# Autodesk Inventor assembly: INDX_000_Main
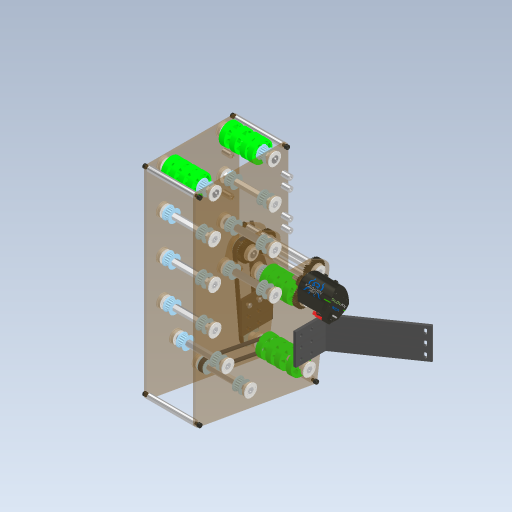
[picture p0: Inventor's stored thumbnail of the model, 512x512]
Saved by Autodesk Inventor 2024 (Build 280153000, 153)
## iProperties
Created: 2024-08-08
Part Number: INDX_000_Main
Document SubType Name: Assembly
Designer: Oscar
Author: Oscar
## Documents named in this file (27)
- C:\Users\Takum\OneDrive\Documents\GitHub\1622-2024-Summer-CAD-A-Thon\Index\INDX_000_Main.iam
- C:\Users\Takum\OneDrive\Documents\GitHub\1622-2024-Summer-CAD-A-Thon\Index\INDX_001_Plate.ipt
- C:\Users\Takum\OneDrive\Documents\GitHub\1622-2024-Summer-CAD-A-Thon\Index\INDX_002_Standoff.ipt
- C:\Users\Takum\OneDrive\Documents\GitHub\1622-2024-Summer-CAD-A-Thon\COTS Library\Motion\Bearings\COTS_WCP-0783_1.125ODHexBearing.ipt
- C:\Users\Takum\OneDrive\Documents\GitHub\1622-2024-Summer-CAD-A-Thon\COTS Library\Motors\COTS_WCP_Full_Kraken.iam
- C:\Users\Takum\OneDrive\Documents\GitHub\1622-2024-Summer-CAD-A-Thon\Index\INDX_003_OuterStandoff.ipt
- C:\Users\Takum\OneDrive\Documents\GitHub\1622-2024-Summer-CAD-A-Thon\Index\INDX_006_Funnel.ipt
- C:\Users\Takum\OneDrive\Documents\GitHub\1622-2024-Summer-CAD-A-Thon\COTS Library\Motion\Gears\Motor Gears\SplineXS\COTS_WCP-1013_14TSplineXsGear.ipt
- C:\Users\Takum\OneDrive\Documents\GitHub\1622-2024-Summer-CAD-A-Thon\COTS Library\Motion\Gears\20DP gears\Steel\0.5in hex\COTS_WCP-0174_Steel_34T20DPGear.ipt
- C:\Users\Takum\OneDrive\Documents\GitHub\1622-2024-Summer-CAD-A-Thon\Index\INDX_007_22TPulley.ipt
- C:\Users\Takum\OneDrive\Documents\GitHub\1622-2024-Summer-CAD-A-Thon\Index\INDX_008_0.5inSpacer.ipt
- C:\Users\Takum\OneDrive\Documents\GitHub\1622-2024-Summer-CAD-A-Thon\COTS Library\Motion\Wheels\Compliant Wheels\2in compliant wheels\0.500in hex bore\COTS_am-3462_2indiameter_0.500inhexbore_durometer35A_CompliantWheel.ipt
- C:\Users\Takum\OneDrive\Documents\GitHub\1622-2024-Summer-CAD-A-Thon\Index\INDX_010_5inHex.ipt
- C:\Users\Takum\OneDrive\Documents\GitHub\1622-2024-Summer-CAD-A-Thon\Index\INDX_011_SecondPlate.ipt
- C:\Users\Takum\OneDrive\Documents\GitHub\1622-2024-Summer-CAD-A-Thon\Index\INDX_012_OuterPlate.ipt
- C:\Users\Takum\OneDrive\Documents\GitHub\1622-2024-Summer-CAD-A-Thon\Index\INDX_013_ThinSpacer.ipt
- C:\Users\Takum\OneDrive\Documents\GitHub\1622-2024-Summer-CAD-A-Thon\Index\INDX_014_Outerstandoff.ipt
- C:\Users\Takum\OneDrive\Documents\GitHub\1622-2024-Summer-CAD-A-Thon\Index\INDX_009_FrontHex.ipt
- C:\Users\Takum\OneDrive\Documents\GitHub\1622-2024-Summer-CAD-A-Thon\Index\INDX_015_OuterHex.ipt
- C:\Users\Takum\OneDrive\Documents\GitHub\1622-2024-Summer-CAD-A-Thon\Index\INDX_016_BottomHex.ipt
- C:\Users\Takum\OneDrive\Documents\GitHub\1622-2024-Summer-CAD-A-Thon\COTS Library\Motion\Pulleys\HTD5M\10mm Wide\COTS_HTD5MM_9mm_16TPulley.ipt
- C:\Users\Takum\OneDrive\Documents\GitHub\1622-2024-Summer-CAD-A-Thon\Index\INDX_017_Mainhex.ipt
- C:\Users\Takum\OneDrive\Documents\GitHub\1622-2024-Summer-CAD-A-Thon\Index\INDX_021_BottomBelt.ipt
- C:\Users\Takum\OneDrive\Documents\GitHub\1622-2024-Summer-CAD-A-Thon\COTS Library\Fasteners\Washers\COTS_90107A029_316 Stainless Steel Washer.ipt
- C:\Users\Takum\OneDrive\Documents\GitHub\1622-2024-Summer-CAD-A-Thon\COTS Library\Fasteners\Bolts\Button-Head\0.25-20\COTS_0.25-20_ButtonHead_0.5inlong_StainlessSteel_92949A537.ipt
- C:\Users\Takum\OneDrive\Documents\GitHub\1622-2024-Summer-CAD-A-Thon\COTS Library\Fasteners\Bolts\Socket-Head\0.25-20\COTS_91251A540_Black-Oxide Alloy Steel Socket Head Screw.ipt
- C:\Users\Takum\OneDrive\Documents\GitHub\1622-2024-Summer-CAD-A-Thon\Index\INDX_022_SideBelt.ipt
## Components (159 placed, 26 different names)
1. INDX_001_Plate:2 — Mate:3, Mate:5, Mate:6, Mate:9, Mate:10, Mate:12, Mate:13, Mate:14, Mate:15, Mate:16, Mate:17, Mate:18, Mate:19, Mate:20, Mate:21, Mate:22, Mate:23, Mate:24, Mate:25, Mate:26, Mate:27, Mate:28, Mate:29, Mate:30, Mate:31, Mate:54, Mate:56, Mate:57, Mate:58, Mate:59, Mate:60, Mate:61, Mate:62, Mate:63, Mate:64, Mate:65, Mate:66, Mate:67, Mate:68, Mate:69, Mate:70, Mate:79, Mate:80, Mate:81, Mate:89, Mate:162, Mate:165, Mate:278, Mate:279, Mate:280, Mate:281, Mate:295, Mate:296, Mate:300, Mate:301
2. INDX_002_Standoff:1 — Mate:9, Mate:149, Mate:274
3. INDX_002_Standoff:2 — Mate:6, Mate:148, Mate:275
4. INDX_002_Standoff:3 — Mate:10, Mate:111, Mate:150
5. INDX_002_Standoff:4 — Mate:3, Mate:5, Mate:110, Mate:112
6. COTS_WCP-0783_1.125ODHexBearing:1 — Mate:18, Mate:19, Mate:264, Mate:265, Mate:311
7. COTS_WCP-0783_1.125ODHexBearing:2 — Mate:16, Mate:17, Mate:310
8. COTS_WCP-0783_1.125ODHexBearing:3 — Mate:20, Mate:21, Mate:318
9. COTS_WCP-0783_1.125ODHexBearing:4 — Mate:22, Mate:23, Mate:262, Mate:263, Mate:319
10. COTS_WCP-0783_1.125ODHexBearing:5 — Mate:13, Mate:14, Mate:307
11. COTS_WCP-0783_1.125ODHexBearing:6 — Mate:12, Mate:15, Mate:306
12. COTS_WCP-0783_1.125ODHexBearing:7 — Mate:24, Mate:25
13. COTS_WCP-0783_1.125ODHexBearing:8 — Mate:26, Mate:27
14. COTS_WCP-0783_1.125ODHexBearing:9 — Mate:30, Mate:31
15. COTS_WCP-0783_1.125ODHexBearing:10 — Mate:28, Mate:29
16. COTS_WCP-0783_1.125ODHexBearing:11 — Mate:140, Mate:141, Mate:194, Flush:11, Mate:216, Mate:217, Mate:308
17. COTS_WCP-0783_1.125ODHexBearing:12 — Mate:132, Mate:133, Mate:192, Flush:9, Mate:218, Mate:313, Mate:316
18. COTS_WCP-0783_1.125ODHexBearing:13 — Mate:134, Mate:135, Mate:242, Flush:16, Mate:288, Mate:317
19. COTS_WCP-0783_1.125ODHexBearing:14 — Mate:146, Mate:147, Mate:189, Flush:6, Mate:198, Mate:202, Mate:203, Mate:302
20. COTS_WCP-0783_1.125ODHexBearing:15 — Mate:130, Mate:131, Mate:191, Flush:8, Mate:212, Mate:314, Mate:315
21. COTS_WCP-0783_1.125ODHexBearing:16 — Mate:142, Mate:143, Mate:193, Flush:10, Mate:214, Mate:215, Mate:305
22. COTS_WCP-0783_1.125ODHexBearing:17 — Mate:144, Mate:145, Mate:190, Flush:7, Mate:204, Mate:205, Mate:303, Mate:304
23. COTS_WCP-0783_1.125ODHexBearing:18 — Mate:96, Mate:100, Mate:102, Mate:153, Mate:154
24. COTS_WCP-0783_1.125ODHexBearing:19 — Mate:138, Mate:139, Mate:196, Flush:13, Mate:286, Mate:309
25. COTS_WCP-0783_1.125ODHexBearing:20 — Mate:113, Mate:114, Mate:195, Flush:12, Mate:250, Mate:260, Mate:261
26. COTS_WCP-0783_1.125ODHexBearing:21 — Mate:136, Mate:137, Mate:197, Flush:14, Mate:254, Mate:258
27. COTS_WCP_Full_Kraken:1 [sub-assembly] — Mate:54, Mate:56, Mate:89, Mate:90
28. COTS_WCP-0783_1.125ODHexBearing:22 — Mate:59, Mate:60, Mate:91, Mate:92
29. COTS_WCP-0783_1.125ODHexBearing:23 — Mate:57, Mate:58, Mate:93, Mate:94
30. COTS_WCP-0783_1.125ODHexBearing:24 — Mate:61, Mate:62, Mate:184
31. INDX_003_OuterStandoff:1 — Mate:115, Mate:116
32. INDX_003_OuterStandoff:2 — Mate:119, Mate:120
33. INDX_003_OuterStandoff:3 — Mate:63, Mate:68
34. INDX_003_OuterStandoff:4 — Mate:64, Mate:69
35. INDX_003_OuterStandoff:5 — Mate:65, Mate:70
36. INDX_003_OuterStandoff:6 — Mate:66, Mate:67
37. INDX_003_OuterStandoff:7 — Mate:117, Mate:118
38. INDX_003_OuterStandoff:8 — Mate:121, Mate:122
39. INDX_006_Funnel:1 — Mate:79, Mate:80, Mate:81
40. INDX_006_Funnel:2 — Mate:123, Mate:124, Mate:125
41. COTS_WCP-0783_1.125ODHexBearing:25 — Mate:126, Mate:127, Mate:128, Mate:129
42. COTS_WCP-0783_1.125ODHexBearing:26 — Mate:109, Flush:2, Mate:151, Mate:152, Mate:210, Mate:312
43. COTS_WCP-1013_14TSplineXsGear:1 — Mate:90
44. COTS_WCP-0174_Steel_34T20DPGear:1 — Mate:93, Mate:94, Mate:108
45. COTS_WCP-0174_Steel_34T20DPGear:2 — Mate:91, Mate:92
46. INDX_007_22TPulley:1 — Mate:159, Mate:160, Mate:172, Mate:173, Mate:248, Mate:249
47. INDX_007_22TPulley:2 — Mate:96, Mate:101, Flush:5, Mate:220, Mate:247
48. INDX_008_0.5inSpacer:1 — Mate:100, Mate:101, Mate:102, Mate:183
49. COTS_am-3462_2indiameter_0.500inhexbore_durometer35A_CompliantWheel:1 — Mate:105
50. COTS_am-3462_2indiameter_0.500inhexbore_durometer35A_CompliantWheel:2 — Mate:106, Mate:107
51. COTS_am-3462_2indiameter_0.500inhexbore_durometer35A_CompliantWheel:3 — Mate:107
52. COTS_am-3462_2indiameter_0.500inhexbore_durometer35A_CompliantWheel:4 — Mate:105, Mate:106, Mate:108
53. INDX_010_5inHex:1 — Mate:109, Flush:2, Mate:211, Mate:234
54. INDX_011_SecondPlate:1 — Mate:110, Mate:111, Mate:112, Mate:113, Mate:114, Mate:115, Mate:116, Mate:117, Mate:118, Mate:119, Mate:120, Mate:121, Mate:122, Mate:123, Mate:124, Mate:125, Mate:126, Mate:127, Mate:130, Mate:131, Mate:132, Mate:133, Mate:134, Mate:135, Mate:136, Mate:137, Mate:138, Mate:139, Mate:140, Mate:141, Mate:142, Mate:143, Mate:144, Mate:145, Mate:146, Mate:147, Mate:148, Mate:149, Mate:150, Mate:151, Mate:152, Mate:153, Mate:154, Mate:155, Mate:156, Mate:157, Mate:163, Mate:164, Mate:166, Mate:167, Mate:175, Mate:177, Mate:179, Mate:243, Mate:244, Mate:245, Mate:246, Mate:276, Mate:277, Mate:294, Mate:297, Mate:298, Mate:299
55. COTS_WCP-0174_Steel_34T20DPGear:3 — Mate:128, Mate:129, Mate:181
56. COTS_WCP-0174_Steel_34T20DPGear:4 — Mate:155, Mate:158, Mate:159, Mate:160
57. COTS_WCP-0783_1.125ODHexBearing:27 — Mate:156, Mate:157, Mate:158, Mate:320
58. INDX_002_Standoff:5 — Mate:162, Mate:163
59. INDX_002_Standoff:6 — Mate:164, Mate:165
60. INDX_012_OuterPlate:1 — Mate:166, Mate:167, Mate:168, Mate:169, Mate:170, Mate:171, Mate:176, Mate:178, Mate:180, Mate:236, Mate:237, Mate:238, Mate:239
61. COTS_WCP-0783_1.125ODHexBearing:28 — Mate:170, Mate:171, Mate:174, Mate:182, Flush:4, Mate:208, Mate:209
62. COTS_WCP-0783_1.125ODHexBearing:29 — Mate:168, Mate:169, Flush:3, Mate:206, Mate:207
63. INDX_013_ThinSpacer:1 — Mate:172, Mate:173, Mate:174
64. INDX_014_Outerstandoff:1 — Mate:175, Mate:176
65. INDX_014_Outerstandoff:2 — Mate:177, Mate:178
66. INDX_014_Outerstandoff:3 — Mate:179, Mate:180
67. INDX_009_FrontHex:1 — Mate:181, Flush:3, Mate:232
68. INDX_015_OuterHex:1 — Mate:182, Flush:4, Mate:230, Mate:321, Mate:322
69. INDX_016_BottomHex:1 — Mate:183, Flush:5, Mate:221, Mate:222
70. COTS_am-3462_2indiameter_0.500inhexbore_durometer35A_CompliantWheel:5 — Mate:184, Mate:185, Mate:186
71. COTS_am-3462_2indiameter_0.500inhexbore_durometer35A_CompliantWheel:6 — Mate:185
72. COTS_am-3462_2indiameter_0.500inhexbore_durometer35A_CompliantWheel:7 — Mate:186, Mate:187, Mate:188
73. COTS_am-3462_2indiameter_0.500inhexbore_durometer35A_CompliantWheel:8 — Mate:187
74. COTS_HTD5MM_9mm_16TPulley:1 — Mate:188, Flush:15, Mate:199
75. INDX_017_Mainhex:1 — Mate:190, Flush:7, Mate:226
76. INDX_017_Mainhex:2 — Mate:189, Flush:6, Mate:224
77. INDX_017_Mainhex:3 — Mate:192, Flush:9, Mate:219, Mate:240
78. INDX_017_Mainhex:4 — Mate:193, Flush:10, Mate:284
79. INDX_017_Mainhex:5 — Mate:191, Flush:8, Mate:213, Mate:228
80. INDX_017_Mainhex:6 — Mate:194, Flush:11, Mate:282
81. INDX_017_Mainhex:7 — Mate:195, Flush:12, Mate:270
82. INDX_017_Mainhex:8 — Mate:196, Flush:13, Mate:287, Mate:292
83. INDX_017_Mainhex:9 — Mate:197, Flush:14, Mate:259, Mate:272
84. COTS_HTD5MM_9mm_16TPulley:2 — Mate:198, Flush:15, Mate:200, Mate:201
85. INDX_021_BottomBelt:1 — Mate:199, Mate:200, Mate:201
86. COTS_90107A029_316 Stainless Steel Washer:1 — Mate:202, Mate:203, Mate:225
87. COTS_90107A029_316 Stainless Steel Washer:2 — Mate:204, Mate:205, Mate:227
88. COTS_90107A029_316 Stainless Steel Washer:3 — Mate:206, Mate:207, Mate:233
89. COTS_90107A029_316 Stainless Steel Washer:4 — Mate:208, Mate:209, Mate:231
90. COTS_90107A029_316 Stainless Steel Washer:5 — Mate:210, Mate:211, Mate:235
91. COTS_90107A029_316 Stainless Steel Washer:6 — Mate:212, Mate:213, Mate:229
92. COTS_90107A029_316 Stainless Steel Washer:7 — Mate:214, Mate:215, Mate:285
93. COTS_90107A029_316 Stainless Steel Washer:8 — Mate:216, Mate:217, Mate:283
94. COTS_90107A029_316 Stainless Steel Washer:9 — Mate:218, Mate:219, Mate:241
95. COTS_0.25-20_ButtonHead_0.5inlong_StainlessSteel_92949A537:1 — Mate:226, Mate:227
96. COTS_0.25-20_ButtonHead_0.5inlong_StainlessSteel_92949A537:2 — Mate:222, Mate:223
97. COTS_0.25-20_ButtonHead_0.5inlong_StainlessSteel_92949A537:3 — Mate:224, Mate:225
98. COTS_90107A029_316 Stainless Steel Washer:10 — Mate:220, Mate:221, Mate:223
99. COTS_0.25-20_ButtonHead_0.5inlong_StainlessSteel_92949A537:4 — Mate:228, Mate:229
100. COTS_0.25-20_ButtonHead_0.5inlong_StainlessSteel_92949A537:5 — Mate:232, Mate:233
101. COTS_0.25-20_ButtonHead_0.5inlong_StainlessSteel_92949A537:6 — Mate:230, Mate:231
102. COTS_0.25-20_ButtonHead_0.5inlong_StainlessSteel_92949A537:7 — Mate:240, Mate:241
103. COTS_0.25-20_ButtonHead_0.5inlong_StainlessSteel_92949A537:8 — Mate:234, Mate:235
104. COTS_91251A540_Black-Oxide Alloy Steel Socket Head Screw:1 — Mate:238, Mate:239
105. COTS_91251A540_Black-Oxide Alloy Steel Socket Head Screw:2 — Mate:236, Mate:237
106. INDX_017_Mainhex:10 — Mate:242, Flush:16, Mate:289, Mate:290
107. COTS_0.25-20_ButtonHead_0.5inlong_StainlessSteel_92949A537:9 — Mate:243, Mate:244
108. COTS_0.25-20_ButtonHead_0.5inlong_StainlessSteel_92949A537:10 — Mate:245, Mate:246
109. COTS_0.25-20_ButtonHead_0.5inlong_StainlessSteel_92949A537:11 — Mate:266, Mate:267
110. INDX_022_SideBelt:1 — Mate:247, Mate:248, Mate:249
111. COTS_am-3462_2indiameter_0.500inhexbore_durometer35A_CompliantWheel:9 — Mate:252, Mate:253
112. COTS_am-3462_2indiameter_0.500inhexbore_durometer35A_CompliantWheel:10 — Mate:253
113. COTS_am-3462_2indiameter_0.500inhexbore_durometer35A_CompliantWheel:11 — Mate:250, Mate:251
114. COTS_am-3462_2indiameter_0.500inhexbore_durometer35A_CompliantWheel:12 — Mate:251, Mate:252
115. COTS_am-3462_2indiameter_0.500inhexbore_durometer35A_CompliantWheel:13 — Mate:255
116. COTS_am-3462_2indiameter_0.500inhexbore_durometer35A_CompliantWheel:14 — Mate:256, Mate:257
117. COTS_am-3462_2indiameter_0.500inhexbore_durometer35A_CompliantWheel:15 — Mate:254, Mate:255, Mate:256
118. COTS_am-3462_2indiameter_0.500inhexbore_durometer35A_CompliantWheel:16 — Mate:257
119. COTS_90107A029_316 Stainless Steel Washer:11 — Mate:258, Mate:259, Mate:273
120. COTS_90107A029_316 Stainless Steel Washer:12 — Mate:260, Mate:261, Mate:271
121. COTS_90107A029_316 Stainless Steel Washer:13 — Mate:264, Mate:265, Mate:268, Mate:269
122. COTS_90107A029_316 Stainless Steel Washer:14 — Mate:262, Mate:263, Mate:266, Mate:267
123. COTS_0.25-20_ButtonHead_0.5inlong_StainlessSteel_92949A537:12 — Mate:270, Mate:271
124. COTS_0.25-20_ButtonHead_0.5inlong_StainlessSteel_92949A537:13 — Mate:272, Mate:273
125. COTS_0.25-20_ButtonHead_0.5inlong_StainlessSteel_92949A537:14 — Mate:268, Mate:269
126. COTS_91251A540_Black-Oxide Alloy Steel Socket Head Screw:3 — Mate:274, Mate:277
127. COTS_91251A540_Black-Oxide Alloy Steel Socket Head Screw:4 — Mate:275, Mate:276
128. COTS_91251A540_Black-Oxide Alloy Steel Socket Head Screw:5 — Mate:280, Mate:281
129. COTS_91251A540_Black-Oxide Alloy Steel Socket Head Screw:6 — Mate:278, Mate:279
130. COTS_0.25-20_ButtonHead_0.5inlong_StainlessSteel_92949A537:15 — Mate:282, Mate:283
131. COTS_0.25-20_ButtonHead_0.5inlong_StainlessSteel_92949A537:16 — Mate:284, Mate:285
132. COTS_90107A029_316 Stainless Steel Washer:15 — Mate:288, Mate:289, Mate:291
133. COTS_90107A029_316 Stainless Steel Washer:16 — Mate:286, Mate:287, Mate:293
134. COTS_0.25-20_ButtonHead_0.5inlong_StainlessSteel_92949A537:17 — Mate:290, Mate:291
135. COTS_0.25-20_ButtonHead_0.5inlong_StainlessSteel_92949A537:18 — Mate:292, Mate:293
136. COTS_91251A540_Black-Oxide Alloy Steel Socket Head Screw:7 — Mate:294, Mate:297
137. COTS_91251A540_Black-Oxide Alloy Steel Socket Head Screw:8 — Mate:295, Mate:296
138. COTS_91251A540_Black-Oxide Alloy Steel Socket Head Screw:9 — Mate:298, Mate:299
139. COTS_91251A540_Black-Oxide Alloy Steel Socket Head Screw:10 — Mate:300, Mate:301
140. COTS_HTD5MM_9mm_16TPulley:3 — Mate:302, Flush:17
141. COTS_HTD5MM_9mm_16TPulley:4 — Mate:303, Flush:17
142. COTS_HTD5MM_9mm_16TPulley:5 — Mate:304, Flush:18
143. COTS_HTD5MM_9mm_16TPulley:6 — Flush:18, Mate:305
144. COTS_HTD5MM_9mm_16TPulley:7 — Mate:306, Flush:19
145. COTS_HTD5MM_9mm_16TPulley:8 — Mate:307, Flush:19
146. COTS_HTD5MM_9mm_16TPulley:9 — Mate:308, Flush:20
147. COTS_HTD5MM_9mm_16TPulley:10 — Mate:309, Flush:20
148. COTS_HTD5MM_9mm_16TPulley:11 — Mate:311, Flush:21
149. COTS_HTD5MM_9mm_16TPulley:12 — Mate:310, Flush:21
150. COTS_HTD5MM_9mm_16TPulley:13 — Mate:313, Flush:23
151. COTS_HTD5MM_9mm_16TPulley:14 — Mate:312, Flush:22
152. COTS_HTD5MM_9mm_16TPulley:15 — Mate:314, Flush:23
153. COTS_HTD5MM_9mm_16TPulley:16 — Mate:315, Flush:22
154. COTS_HTD5MM_9mm_16TPulley:17 — Mate:318, Flush:25
155. COTS_HTD5MM_9mm_16TPulley:18 — Mate:319, Flush:25
156. COTS_HTD5MM_9mm_16TPulley:19 — Mate:316, Flush:24
157. COTS_HTD5MM_9mm_16TPulley:20 — Mate:317, Flush:24
158. COTS_90107A029_316 Stainless Steel Washer:17 — Mate:320, Mate:321, Mate:323
159. COTS_0.25-20_ButtonHead_0.5inlong_StainlessSteel_92949A537:19 — Mate:322, Mate:323
## Relationships (296: Mate 272, Flush 24)
- Mate:3: INDX_001_Plate:2 ↔ INDX_002_Standoff:4
- Mate:5: INDX_001_Plate:2 ↔ INDX_002_Standoff:4
- Mate:6: INDX_001_Plate:2 ↔ INDX_002_Standoff:2
- Mate:9: INDX_001_Plate:2 ↔ INDX_002_Standoff:1
- Mate:10: INDX_001_Plate:2 ↔ INDX_002_Standoff:3
- Mate:12: INDX_001_Plate:2 ↔ COTS_WCP-0783_1.125ODHexBearing:6
- Mate:13: INDX_001_Plate:2 ↔ COTS_WCP-0783_1.125ODHexBearing:5
- Mate:14: INDX_001_Plate:2 ↔ COTS_WCP-0783_1.125ODHexBearing:5
- Mate:15: INDX_001_Plate:2 ↔ COTS_WCP-0783_1.125ODHexBearing:6
- Mate:16: INDX_001_Plate:2 ↔ COTS_WCP-0783_1.125ODHexBearing:2
- Mate:17: INDX_001_Plate:2 ↔ COTS_WCP-0783_1.125ODHexBearing:2
- Mate:18: INDX_001_Plate:2 ↔ COTS_WCP-0783_1.125ODHexBearing:1
- Mate:19: INDX_001_Plate:2 ↔ COTS_WCP-0783_1.125ODHexBearing:1
- Mate:20: INDX_001_Plate:2 ↔ COTS_WCP-0783_1.125ODHexBearing:3
- Mate:21: INDX_001_Plate:2 ↔ COTS_WCP-0783_1.125ODHexBearing:3
- Mate:22: INDX_001_Plate:2 ↔ COTS_WCP-0783_1.125ODHexBearing:4
- Mate:23: INDX_001_Plate:2 ↔ COTS_WCP-0783_1.125ODHexBearing:4
- Mate:24: INDX_001_Plate:2 ↔ COTS_WCP-0783_1.125ODHexBearing:7
- Mate:25: INDX_001_Plate:2 ↔ COTS_WCP-0783_1.125ODHexBearing:7
- Mate:26: INDX_001_Plate:2 ↔ COTS_WCP-0783_1.125ODHexBearing:8
- Mate:27: INDX_001_Plate:2 ↔ COTS_WCP-0783_1.125ODHexBearing:8
- Mate:28: INDX_001_Plate:2 ↔ COTS_WCP-0783_1.125ODHexBearing:10
- Mate:29: INDX_001_Plate:2 ↔ COTS_WCP-0783_1.125ODHexBearing:10
- Mate:30: INDX_001_Plate:2 ↔ COTS_WCP-0783_1.125ODHexBearing:9
- Mate:31: INDX_001_Plate:2 ↔ COTS_WCP-0783_1.125ODHexBearing:9
- Mate:54: INDX_001_Plate:2 ↔ COTS_WCP_Full_Kraken:1
- Mate:56: INDX_001_Plate:2 ↔ COTS_WCP_Full_Kraken:1
- Mate:57: INDX_001_Plate:2 ↔ COTS_WCP-0783_1.125ODHexBearing:23
- Mate:58: INDX_001_Plate:2 ↔ COTS_WCP-0783_1.125ODHexBearing:23
- Mate:59: INDX_001_Plate:2 ↔ COTS_WCP-0783_1.125ODHexBearing:22
- Mate:60: INDX_001_Plate:2 ↔ COTS_WCP-0783_1.125ODHexBearing:22
- Mate:61: INDX_001_Plate:2 ↔ COTS_WCP-0783_1.125ODHexBearing:24
- Mate:62: INDX_001_Plate:2 ↔ COTS_WCP-0783_1.125ODHexBearing:24
- Mate:63: INDX_001_Plate:2 ↔ INDX_003_OuterStandoff:3
- Mate:64: INDX_001_Plate:2 ↔ INDX_003_OuterStandoff:4
- Mate:65: INDX_001_Plate:2 ↔ INDX_003_OuterStandoff:5
- Mate:66: INDX_001_Plate:2 ↔ INDX_003_OuterStandoff:6
- Mate:67: INDX_001_Plate:2 ↔ INDX_003_OuterStandoff:6
- Mate:68: INDX_001_Plate:2 ↔ INDX_003_OuterStandoff:3
- Mate:69: INDX_001_Plate:2 ↔ INDX_003_OuterStandoff:4
- Mate:70: INDX_001_Plate:2 ↔ INDX_003_OuterStandoff:5
- Mate:79: INDX_001_Plate:2 ↔ INDX_006_Funnel:1
- Mate:80: INDX_001_Plate:2 ↔ INDX_006_Funnel:1
- Mate:81: INDX_001_Plate:2 ↔ INDX_006_Funnel:1
- Mate:89: INDX_001_Plate:2 ↔ COTS_WCP_Full_Kraken:1
- Mate:90: COTS_WCP_Full_Kraken:1 ↔ COTS_WCP-1013_14TSplineXsGear:1
- Mate:91: COTS_WCP-0783_1.125ODHexBearing:22 ↔ COTS_WCP-0174_Steel_34T20DPGear:2
- Mate:92: COTS_WCP-0783_1.125ODHexBearing:22 ↔ COTS_WCP-0174_Steel_34T20DPGear:2
- Mate:93: COTS_WCP-0783_1.125ODHexBearing:23 ↔ COTS_WCP-0174_Steel_34T20DPGear:1
- Mate:94: COTS_WCP-0783_1.125ODHexBearing:23 ↔ COTS_WCP-0174_Steel_34T20DPGear:1
- Mate:96: COTS_WCP-0783_1.125ODHexBearing:18 ↔ INDX_007_22TPulley:2
- Mate:100: COTS_WCP-0783_1.125ODHexBearing:18 ↔ INDX_008_0.5inSpacer:1
- Mate:101: INDX_007_22TPulley:2 ↔ INDX_008_0.5inSpacer:1
- Mate:102: COTS_WCP-0783_1.125ODHexBearing:18 ↔ INDX_008_0.5inSpacer:1
- Mate:105: COTS_am-3462_2indiameter_0.500inhexbore_durometer35A_CompliantWheel:1 ↔ COTS_am-3462_2indiameter_0.500inhexbore_durometer35A_CompliantWheel:4
- Mate:106: COTS_am-3462_2indiameter_0.500inhexbore_durometer35A_CompliantWheel:2 ↔ COTS_am-3462_2indiameter_0.500inhexbore_durometer35A_CompliantWheel:4
- Mate:107: COTS_am-3462_2indiameter_0.500inhexbore_durometer35A_CompliantWheel:2 ↔ COTS_am-3462_2indiameter_0.500inhexbore_durometer35A_CompliantWheel:3
- Mate:108: COTS_WCP-0174_Steel_34T20DPGear:1 ↔ COTS_am-3462_2indiameter_0.500inhexbore_durometer35A_CompliantWheel:4
- Mate:109: COTS_WCP-0783_1.125ODHexBearing:26 ↔ INDX_010_5inHex:1
- Flush:2: COTS_WCP-0783_1.125ODHexBearing:26 ↔ INDX_010_5inHex:1
- Mate:110: INDX_002_Standoff:4 ↔ INDX_011_SecondPlate:1
- Mate:111: INDX_002_Standoff:3 ↔ INDX_011_SecondPlate:1
- Mate:112: INDX_002_Standoff:4 ↔ INDX_011_SecondPlate:1
- Mate:113: COTS_WCP-0783_1.125ODHexBearing:20 ↔ INDX_011_SecondPlate:1
- Mate:114: COTS_WCP-0783_1.125ODHexBearing:20 ↔ INDX_011_SecondPlate:1
- Mate:115: INDX_003_OuterStandoff:1 ↔ INDX_011_SecondPlate:1
- Mate:116: INDX_003_OuterStandoff:1 ↔ INDX_011_SecondPlate:1
- Mate:117: INDX_003_OuterStandoff:7 ↔ INDX_011_SecondPlate:1
- Mate:118: INDX_003_OuterStandoff:7 ↔ INDX_011_SecondPlate:1
- Mate:119: INDX_003_OuterStandoff:2 ↔ INDX_011_SecondPlate:1
- Mate:120: INDX_003_OuterStandoff:2 ↔ INDX_011_SecondPlate:1
- Mate:121: INDX_003_OuterStandoff:8 ↔ INDX_011_SecondPlate:1
- Mate:122: INDX_003_OuterStandoff:8 ↔ INDX_011_SecondPlate:1
- Mate:123: INDX_006_Funnel:2 ↔ INDX_011_SecondPlate:1
- Mate:124: INDX_006_Funnel:2 ↔ INDX_011_SecondPlate:1
- Mate:125: INDX_006_Funnel:2 ↔ INDX_011_SecondPlate:1
- Mate:126: COTS_WCP-0783_1.125ODHexBearing:25 ↔ INDX_011_SecondPlate:1
- Mate:127: COTS_WCP-0783_1.125ODHexBearing:25 ↔ INDX_011_SecondPlate:1
- Mate:128: COTS_WCP-0783_1.125ODHexBearing:25 ↔ COTS_WCP-0174_Steel_34T20DPGear:3
- Mate:129: COTS_WCP-0783_1.125ODHexBearing:25 ↔ COTS_WCP-0174_Steel_34T20DPGear:3
- Mate:130: COTS_WCP-0783_1.125ODHexBearing:15 ↔ INDX_011_SecondPlate:1
- Mate:131: COTS_WCP-0783_1.125ODHexBearing:15 ↔ INDX_011_SecondPlate:1
- Mate:132: COTS_WCP-0783_1.125ODHexBearing:12 ↔ INDX_011_SecondPlate:1
- Mate:133: COTS_WCP-0783_1.125ODHexBearing:12 ↔ INDX_011_SecondPlate:1
- Mate:134: COTS_WCP-0783_1.125ODHexBearing:13 ↔ INDX_011_SecondPlate:1
- Mate:135: COTS_WCP-0783_1.125ODHexBearing:13 ↔ INDX_011_SecondPlate:1
- Mate:136: COTS_WCP-0783_1.125ODHexBearing:21 ↔ INDX_011_SecondPlate:1
- Mate:137: COTS_WCP-0783_1.125ODHexBearing:21 ↔ INDX_011_SecondPlate:1
- Mate:138: COTS_WCP-0783_1.125ODHexBearing:19 ↔ INDX_011_SecondPlate:1
- Mate:139: COTS_WCP-0783_1.125ODHexBearing:19 ↔ INDX_011_SecondPlate:1
- Mate:140: COTS_WCP-0783_1.125ODHexBearing:11 ↔ INDX_011_SecondPlate:1
- Mate:141: COTS_WCP-0783_1.125ODHexBearing:11 ↔ INDX_011_SecondPlate:1
- Mate:142: COTS_WCP-0783_1.125ODHexBearing:16 ↔ INDX_011_SecondPlate:1
- Mate:143: COTS_WCP-0783_1.125ODHexBearing:16 ↔ INDX_011_SecondPlate:1
- Mate:144: COTS_WCP-0783_1.125ODHexBearing:17 ↔ INDX_011_SecondPlate:1
- Mate:145: COTS_WCP-0783_1.125ODHexBearing:17 ↔ INDX_011_SecondPlate:1
- Mate:146: COTS_WCP-0783_1.125ODHexBearing:14 ↔ INDX_011_SecondPlate:1
- Mate:147: COTS_WCP-0783_1.125ODHexBearing:14 ↔ INDX_011_SecondPlate:1
- Mate:148: INDX_002_Standoff:2 ↔ INDX_011_SecondPlate:1
- Mate:149: INDX_002_Standoff:1 ↔ INDX_011_SecondPlate:1
- Mate:150: INDX_002_Standoff:3 ↔ INDX_011_SecondPlate:1
- Mate:151: COTS_WCP-0783_1.125ODHexBearing:26 ↔ INDX_011_SecondPlate:1
- Mate:152: COTS_WCP-0783_1.125ODHexBearing:26 ↔ INDX_011_SecondPlate:1
- Mate:153: COTS_WCP-0783_1.125ODHexBearing:18 ↔ INDX_011_SecondPlate:1
- Mate:154: COTS_WCP-0783_1.125ODHexBearing:18 ↔ INDX_011_SecondPlate:1
- Mate:155: INDX_011_SecondPlate:1 ↔ COTS_WCP-0174_Steel_34T20DPGear:4
- Mate:156: INDX_011_SecondPlate:1 ↔ COTS_WCP-0783_1.125ODHexBearing:27
- Mate:157: INDX_011_SecondPlate:1 ↔ COTS_WCP-0783_1.125ODHexBearing:27
- Mate:158: COTS_WCP-0174_Steel_34T20DPGear:4 ↔ COTS_WCP-0783_1.125ODHexBearing:27
- Mate:159: INDX_007_22TPulley:1 ↔ COTS_WCP-0174_Steel_34T20DPGear:4
- Mate:160: INDX_007_22TPulley:1 ↔ COTS_WCP-0174_Steel_34T20DPGear:4
- Mate:162: INDX_001_Plate:2 ↔ INDX_002_Standoff:5
- Mate:163: INDX_011_SecondPlate:1 ↔ INDX_002_Standoff:5
- Mate:164: INDX_011_SecondPlate:1 ↔ INDX_002_Standoff:6
- Mate:165: INDX_001_Plate:2 ↔ INDX_002_Standoff:6
- Mate:166: INDX_011_SecondPlate:1 ↔ INDX_012_OuterPlate:1
- Mate:167: INDX_011_SecondPlate:1 ↔ INDX_012_OuterPlate:1
- Mate:168: INDX_012_OuterPlate:1 ↔ COTS_WCP-0783_1.125ODHexBearing:29
- Mate:169: INDX_012_OuterPlate:1 ↔ COTS_WCP-0783_1.125ODHexBearing:29
- Mate:170: INDX_012_OuterPlate:1 ↔ COTS_WCP-0783_1.125ODHexBearing:28
- Mate:171: INDX_012_OuterPlate:1 ↔ COTS_WCP-0783_1.125ODHexBearing:28
- Mate:172: INDX_007_22TPulley:1 ↔ INDX_013_ThinSpacer:1
- Mate:173: INDX_007_22TPulley:1 ↔ INDX_013_ThinSpacer:1
- Mate:174: COTS_WCP-0783_1.125ODHexBearing:28 ↔ INDX_013_ThinSpacer:1
- Mate:175: INDX_011_SecondPlate:1 ↔ INDX_014_Outerstandoff:1
- Mate:176: INDX_012_OuterPlate:1 ↔ INDX_014_Outerstandoff:1
- Mate:177: INDX_011_SecondPlate:1 ↔ INDX_014_Outerstandoff:2
- Mate:178: INDX_012_OuterPlate:1 ↔ INDX_014_Outerstandoff:2
- Mate:179: INDX_011_SecondPlate:1 ↔ INDX_014_Outerstandoff:3
- Mate:180: INDX_012_OuterPlate:1 ↔ INDX_014_Outerstandoff:3
- Mate:181: COTS_WCP-0174_Steel_34T20DPGear:3 ↔ INDX_009_FrontHex:1
- Flush:3: COTS_WCP-0783_1.125ODHexBearing:29 ↔ INDX_009_FrontHex:1
- Mate:182: COTS_WCP-0783_1.125ODHexBearing:28 ↔ INDX_015_OuterHex:1
- Flush:4: COTS_WCP-0783_1.125ODHexBearing:28 ↔ INDX_015_OuterHex:1
- Mate:183: INDX_008_0.5inSpacer:1 ↔ INDX_016_BottomHex:1
- Flush:5: INDX_007_22TPulley:2 ↔ INDX_016_BottomHex:1
- Mate:184: COTS_WCP-0783_1.125ODHexBearing:24 ↔ COTS_am-3462_2indiameter_0.500inhexbore_durometer35A_CompliantWheel:5
- Mate:185: COTS_am-3462_2indiameter_0.500inhexbore_durometer35A_CompliantWheel:5 ↔ COTS_am-3462_2indiameter_0.500inhexbore_durometer35A_CompliantWheel:6
- Mate:186: COTS_am-3462_2indiameter_0.500inhexbore_durometer35A_CompliantWheel:5 ↔ COTS_am-3462_2indiameter_0.500inhexbore_durometer35A_CompliantWheel:7
- Mate:187: COTS_am-3462_2indiameter_0.500inhexbore_durometer35A_CompliantWheel:7 ↔ COTS_am-3462_2indiameter_0.500inhexbore_durometer35A_CompliantWheel:8
- Mate:188: COTS_am-3462_2indiameter_0.500inhexbore_durometer35A_CompliantWheel:7 ↔ COTS_HTD5MM_9mm_16TPulley:1
- Mate:189: COTS_WCP-0783_1.125ODHexBearing:14 ↔ INDX_017_Mainhex:2
- Flush:6: COTS_WCP-0783_1.125ODHexBearing:14 ↔ INDX_017_Mainhex:2
- Mate:190: COTS_WCP-0783_1.125ODHexBearing:17 ↔ INDX_017_Mainhex:1
- Flush:7: COTS_WCP-0783_1.125ODHexBearing:17 ↔ INDX_017_Mainhex:1
- Mate:191: COTS_WCP-0783_1.125ODHexBearing:15 ↔ INDX_017_Mainhex:5
- Flush:8: COTS_WCP-0783_1.125ODHexBearing:15 ↔ INDX_017_Mainhex:5
- Mate:192: COTS_WCP-0783_1.125ODHexBearing:12 ↔ INDX_017_Mainhex:3
- Flush:9: COTS_WCP-0783_1.125ODHexBearing:12 ↔ INDX_017_Mainhex:3
- Mate:193: COTS_WCP-0783_1.125ODHexBearing:16 ↔ INDX_017_Mainhex:4
- Flush:10: COTS_WCP-0783_1.125ODHexBearing:16 ↔ INDX_017_Mainhex:4
- Mate:194: COTS_WCP-0783_1.125ODHexBearing:11 ↔ INDX_017_Mainhex:6
- Flush:11: COTS_WCP-0783_1.125ODHexBearing:11 ↔ INDX_017_Mainhex:6
- Mate:195: COTS_WCP-0783_1.125ODHexBearing:20 ↔ INDX_017_Mainhex:7
- Flush:12: COTS_WCP-0783_1.125ODHexBearing:20 ↔ INDX_017_Mainhex:7
- Mate:196: COTS_WCP-0783_1.125ODHexBearing:19 ↔ INDX_017_Mainhex:8
- Flush:13: COTS_WCP-0783_1.125ODHexBearing:19 ↔ INDX_017_Mainhex:8
- Mate:197: COTS_WCP-0783_1.125ODHexBearing:21 ↔ INDX_017_Mainhex:9
- Flush:14: COTS_WCP-0783_1.125ODHexBearing:21 ↔ INDX_017_Mainhex:9
- Mate:198: COTS_WCP-0783_1.125ODHexBearing:14 ↔ COTS_HTD5MM_9mm_16TPulley:2
- Flush:15: COTS_HTD5MM_9mm_16TPulley:1 ↔ COTS_HTD5MM_9mm_16TPulley:2
- Mate:199: COTS_HTD5MM_9mm_16TPulley:1 ↔ INDX_021_BottomBelt:1
- Mate:200: COTS_HTD5MM_9mm_16TPulley:2 ↔ INDX_021_BottomBelt:1
- Mate:201 (1 mm): COTS_HTD5MM_9mm_16TPulley:2 ↔ INDX_021_BottomBelt:1
- Mate:202: COTS_WCP-0783_1.125ODHexBearing:14 ↔ COTS_90107A029_316 Stainless Steel Washer:1
- Mate:203: COTS_WCP-0783_1.125ODHexBearing:14 ↔ COTS_90107A029_316 Stainless Steel Washer:1
- Mate:204: COTS_WCP-0783_1.125ODHexBearing:17 ↔ COTS_90107A029_316 Stainless Steel Washer:2
- Mate:205: COTS_WCP-0783_1.125ODHexBearing:17 ↔ COTS_90107A029_316 Stainless Steel Washer:2
- Mate:206: COTS_WCP-0783_1.125ODHexBearing:29 ↔ COTS_90107A029_316 Stainless Steel Washer:3
- Mate:207: COTS_WCP-0783_1.125ODHexBearing:29 ↔ COTS_90107A029_316 Stainless Steel Washer:3
- Mate:208: COTS_WCP-0783_1.125ODHexBearing:28 ↔ COTS_90107A029_316 Stainless Steel Washer:4
- Mate:209: COTS_WCP-0783_1.125ODHexBearing:28 ↔ COTS_90107A029_316 Stainless Steel Washer:4
- Mate:210: COTS_WCP-0783_1.125ODHexBearing:26 ↔ COTS_90107A029_316 Stainless Steel Washer:5
- Mate:211: INDX_010_5inHex:1 ↔ COTS_90107A029_316 Stainless Steel Washer:5
- Mate:212: COTS_WCP-0783_1.125ODHexBearing:15 ↔ COTS_90107A029_316 Stainless Steel Washer:6
- Mate:213: INDX_017_Mainhex:5 ↔ COTS_90107A029_316 Stainless Steel Washer:6
- Mate:214: COTS_WCP-0783_1.125ODHexBearing:16 ↔ COTS_90107A029_316 Stainless Steel Washer:7
- Mate:215: COTS_WCP-0783_1.125ODHexBearing:16 ↔ COTS_90107A029_316 Stainless Steel Washer:7
- Mate:216: COTS_WCP-0783_1.125ODHexBearing:11 ↔ COTS_90107A029_316 Stainless Steel Washer:8
- Mate:217: COTS_WCP-0783_1.125ODHexBearing:11 ↔ COTS_90107A029_316 Stainless Steel Washer:8
- Mate:218: COTS_WCP-0783_1.125ODHexBearing:12 ↔ COTS_90107A029_316 Stainless Steel Washer:9
- Mate:219: INDX_017_Mainhex:3 ↔ COTS_90107A029_316 Stainless Steel Washer:9
- Mate:220: INDX_007_22TPulley:2 ↔ COTS_90107A029_316 Stainless Steel Washer:10
- Mate:221: INDX_016_BottomHex:1 ↔ COTS_90107A029_316 Stainless Steel Washer:10
- Mate:222: INDX_016_BottomHex:1 ↔ COTS_0.25-20_ButtonHead_0.5inlong_StainlessSteel_92949A537:2
- Mate:223: COTS_0.25-20_ButtonHead_0.5inlong_StainlessSteel_92949A537:2 ↔ COTS_90107A029_316 Stainless Steel Washer:10
- Mate:224: INDX_017_Mainhex:2 ↔ COTS_0.25-20_ButtonHead_0.5inlong_StainlessSteel_92949A537:3
- Mate:225: COTS_90107A029_316 Stainless Steel Washer:1 ↔ COTS_0.25-20_ButtonHead_0.5inlong_StainlessSteel_92949A537:3
- Mate:226: INDX_017_Mainhex:1 ↔ COTS_0.25-20_ButtonHead_0.5inlong_StainlessSteel_92949A537:1
- Mate:227: COTS_90107A029_316 Stainless Steel Washer:2 ↔ COTS_0.25-20_ButtonHead_0.5inlong_StainlessSteel_92949A537:1
- Mate:228: INDX_017_Mainhex:5 ↔ COTS_0.25-20_ButtonHead_0.5inlong_StainlessSteel_92949A537:4
- Mate:229: COTS_90107A029_316 Stainless Steel Washer:6 ↔ COTS_0.25-20_ButtonHead_0.5inlong_StainlessSteel_92949A537:4
- Mate:230: INDX_015_OuterHex:1 ↔ COTS_0.25-20_ButtonHead_0.5inlong_StainlessSteel_92949A537:6
- Mate:231: COTS_90107A029_316 Stainless Steel Washer:4 ↔ COTS_0.25-20_ButtonHead_0.5inlong_StainlessSteel_92949A537:6
- Mate:232: INDX_009_FrontHex:1 ↔ COTS_0.25-20_ButtonHead_0.5inlong_StainlessSteel_92949A537:5
- Mate:233: COTS_90107A029_316 Stainless Steel Washer:3 ↔ COTS_0.25-20_ButtonHead_0.5inlong_StainlessSteel_92949A537:5
- Mate:234: INDX_010_5inHex:1 ↔ COTS_0.25-20_ButtonHead_0.5inlong_StainlessSteel_92949A537:8
- Mate:235: COTS_90107A029_316 Stainless Steel Washer:5 ↔ COTS_0.25-20_ButtonHead_0.5inlong_StainlessSteel_92949A537:8
- Mate:236: INDX_012_OuterPlate:1 ↔ COTS_91251A540_Black-Oxide Alloy Steel Socket Head Screw:2
- Mate:237: INDX_012_OuterPlate:1 ↔ COTS_91251A540_Black-Oxide Alloy Steel Socket Head Screw:2
- Mate:238: INDX_012_OuterPlate:1 ↔ COTS_91251A540_Black-Oxide Alloy Steel Socket Head Screw:1
- Mate:239: INDX_012_OuterPlate:1 ↔ COTS_91251A540_Black-Oxide Alloy Steel Socket Head Screw:1
- Mate:240: INDX_017_Mainhex:3 ↔ COTS_0.25-20_ButtonHead_0.5inlong_StainlessSteel_92949A537:7
- Mate:241: COTS_90107A029_316 Stainless Steel Washer:9 ↔ COTS_0.25-20_ButtonHead_0.5inlong_StainlessSteel_92949A537:7
- Mate:242: COTS_WCP-0783_1.125ODHexBearing:13 ↔ INDX_017_Mainhex:10
- Flush:16: COTS_WCP-0783_1.125ODHexBearing:13 ↔ INDX_017_Mainhex:10
- Mate:243: INDX_011_SecondPlate:1 ↔ COTS_0.25-20_ButtonHead_0.5inlong_StainlessSteel_92949A537:9
- Mate:244: INDX_011_SecondPlate:1 ↔ COTS_0.25-20_ButtonHead_0.5inlong_StainlessSteel_92949A537:9
- Mate:245: INDX_011_SecondPlate:1 ↔ COTS_0.25-20_ButtonHead_0.5inlong_StainlessSteel_92949A537:10
- Mate:246: INDX_011_SecondPlate:1 ↔ COTS_0.25-20_ButtonHead_0.5inlong_StainlessSteel_92949A537:10
- Mate:247: INDX_007_22TPulley:2 ↔ INDX_022_SideBelt:1
- Mate:248: INDX_007_22TPulley:1 ↔ INDX_022_SideBelt:1
- Mate:249 (0.5 mm): INDX_007_22TPulley:1 ↔ INDX_022_SideBelt:1
- Mate:250: COTS_WCP-0783_1.125ODHexBearing:20 ↔ COTS_am-3462_2indiameter_0.500inhexbore_durometer35A_CompliantWheel:11
- Mate:251: COTS_am-3462_2indiameter_0.500inhexbore_durometer35A_CompliantWheel:11 ↔ COTS_am-3462_2indiameter_0.500inhexbore_durometer35A_CompliantWheel:12
- Mate:252: COTS_am-3462_2indiameter_0.500inhexbore_durometer35A_CompliantWheel:9 ↔ COTS_am-3462_2indiameter_0.500inhexbore_durometer35A_CompliantWheel:12
- Mate:253: COTS_am-3462_2indiameter_0.500inhexbore_durometer35A_CompliantWheel:9 ↔ COTS_am-3462_2indiameter_0.500inhexbore_durometer35A_CompliantWheel:10
- Mate:254: COTS_WCP-0783_1.125ODHexBearing:21 ↔ COTS_am-3462_2indiameter_0.500inhexbore_durometer35A_CompliantWheel:15
- Mate:255: COTS_am-3462_2indiameter_0.500inhexbore_durometer35A_CompliantWheel:13 ↔ COTS_am-3462_2indiameter_0.500inhexbore_durometer35A_CompliantWheel:15
- Mate:256: COTS_am-3462_2indiameter_0.500inhexbore_durometer35A_CompliantWheel:14 ↔ COTS_am-3462_2indiameter_0.500inhexbore_durometer35A_CompliantWheel:15
- Mate:257: COTS_am-3462_2indiameter_0.500inhexbore_durometer35A_CompliantWheel:14 ↔ COTS_am-3462_2indiameter_0.500inhexbore_durometer35A_CompliantWheel:16
- Mate:258: COTS_WCP-0783_1.125ODHexBearing:21 ↔ COTS_90107A029_316 Stainless Steel Washer:11
- Mate:259: INDX_017_Mainhex:9 ↔ COTS_90107A029_316 Stainless Steel Washer:11
- Mate:260: COTS_WCP-0783_1.125ODHexBearing:20 ↔ COTS_90107A029_316 Stainless Steel Washer:12
- Mate:261: COTS_WCP-0783_1.125ODHexBearing:20 ↔ COTS_90107A029_316 Stainless Steel Washer:12
- Mate:262: COTS_WCP-0783_1.125ODHexBearing:4 ↔ COTS_90107A029_316 Stainless Steel Washer:14
- Mate:263: COTS_WCP-0783_1.125ODHexBearing:4 ↔ COTS_90107A029_316 Stainless Steel Washer:14
- Mate:264: COTS_WCP-0783_1.125ODHexBearing:1 ↔ COTS_90107A029_316 Stainless Steel Washer:13
- Mate:265: COTS_WCP-0783_1.125ODHexBearing:1 ↔ COTS_90107A029_316 Stainless Steel Washer:13
- Mate:266: COTS_0.25-20_ButtonHead_0.5inlong_StainlessSteel_92949A537:11 ↔ COTS_90107A029_316 Stainless Steel Washer:14
- Mate:267: COTS_0.25-20_ButtonHead_0.5inlong_StainlessSteel_92949A537:11 ↔ COTS_90107A029_316 Stainless Steel Washer:14
- Mate:268: COTS_90107A029_316 Stainless Steel Washer:13 ↔ COTS_0.25-20_ButtonHead_0.5inlong_StainlessSteel_92949A537:14
- Mate:269: COTS_90107A029_316 Stainless Steel Washer:13 ↔ COTS_0.25-20_ButtonHead_0.5inlong_StainlessSteel_92949A537:14
- Mate:270: INDX_017_Mainhex:7 ↔ COTS_0.25-20_ButtonHead_0.5inlong_StainlessSteel_92949A537:12
- Mate:271: COTS_90107A029_316 Stainless Steel Washer:12 ↔ COTS_0.25-20_ButtonHead_0.5inlong_StainlessSteel_92949A537:12
- Mate:272: INDX_017_Mainhex:9 ↔ COTS_0.25-20_ButtonHead_0.5inlong_StainlessSteel_92949A537:13
- Mate:273: COTS_90107A029_316 Stainless Steel Washer:11 ↔ COTS_0.25-20_ButtonHead_0.5inlong_StainlessSteel_92949A537:13
- Mate:274: INDX_002_Standoff:1 ↔ COTS_91251A540_Black-Oxide Alloy Steel Socket Head Screw:3
- Mate:275: INDX_002_Standoff:2 ↔ COTS_91251A540_Black-Oxide Alloy Steel Socket Head Screw:4
- Mate:276: INDX_011_SecondPlate:1 ↔ COTS_91251A540_Black-Oxide Alloy Steel Socket Head Screw:4
- Mate:277: INDX_011_SecondPlate:1 ↔ COTS_91251A540_Black-Oxide Alloy Steel Socket Head Screw:3
- Mate:278: INDX_001_Plate:2 ↔ COTS_91251A540_Black-Oxide Alloy Steel Socket Head Screw:6
- Mate:279: INDX_001_Plate:2 ↔ COTS_91251A540_Black-Oxide Alloy Steel Socket Head Screw:6
- Mate:280: INDX_001_Plate:2 ↔ COTS_91251A540_Black-Oxide Alloy Steel Socket Head Screw:5
- Mate:281: INDX_001_Plate:2 ↔ COTS_91251A540_Black-Oxide Alloy Steel Socket Head Screw:5
- Mate:282: INDX_017_Mainhex:6 ↔ COTS_0.25-20_ButtonHead_0.5inlong_StainlessSteel_92949A537:15
- Mate:283: COTS_90107A029_316 Stainless Steel Washer:8 ↔ COTS_0.25-20_ButtonHead_0.5inlong_StainlessSteel_92949A537:15
- Mate:284: INDX_017_Mainhex:4 ↔ COTS_0.25-20_ButtonHead_0.5inlong_StainlessSteel_92949A537:16
- Mate:285: COTS_90107A029_316 Stainless Steel Washer:7 ↔ COTS_0.25-20_ButtonHead_0.5inlong_StainlessSteel_92949A537:16
- Mate:286: COTS_WCP-0783_1.125ODHexBearing:19 ↔ COTS_90107A029_316 Stainless Steel Washer:16
- Mate:287: INDX_017_Mainhex:8 ↔ COTS_90107A029_316 Stainless Steel Washer:16
- Mate:288: COTS_WCP-0783_1.125ODHexBearing:13 ↔ COTS_90107A029_316 Stainless Steel Washer:15
- Mate:289: INDX_017_Mainhex:10 ↔ COTS_90107A029_316 Stainless Steel Washer:15
- Mate:290: INDX_017_Mainhex:10 ↔ COTS_0.25-20_ButtonHead_0.5inlong_StainlessSteel_92949A537:17
- Mate:291: COTS_90107A029_316 Stainless Steel Washer:15 ↔ COTS_0.25-20_ButtonHead_0.5inlong_StainlessSteel_92949A537:17
- Mate:292: INDX_017_Mainhex:8 ↔ COTS_0.25-20_ButtonHead_0.5inlong_StainlessSteel_92949A537:18
- Mate:293: COTS_90107A029_316 Stainless Steel Washer:16 ↔ COTS_0.25-20_ButtonHead_0.5inlong_StainlessSteel_92949A537:18
- Mate:294: INDX_011_SecondPlate:1 ↔ COTS_91251A540_Black-Oxide Alloy Steel Socket Head Screw:7
- Mate:295: INDX_001_Plate:2 ↔ COTS_91251A540_Black-Oxide Alloy Steel Socket Head Screw:8
- Mate:296: INDX_001_Plate:2 ↔ COTS_91251A540_Black-Oxide Alloy Steel Socket Head Screw:8
- Mate:297: INDX_011_SecondPlate:1 ↔ COTS_91251A540_Black-Oxide Alloy Steel Socket Head Screw:7
- Mate:298: INDX_011_SecondPlate:1 ↔ COTS_91251A540_Black-Oxide Alloy Steel Socket Head Screw:9
- Mate:299: INDX_011_SecondPlate:1 ↔ COTS_91251A540_Black-Oxide Alloy Steel Socket Head Screw:9
- Mate:300: INDX_001_Plate:2 ↔ COTS_91251A540_Black-Oxide Alloy Steel Socket Head Screw:10
- Mate:301: INDX_001_Plate:2 ↔ COTS_91251A540_Black-Oxide Alloy Steel Socket Head Screw:10
- Mate:302: COTS_WCP-0783_1.125ODHexBearing:14 ↔ COTS_HTD5MM_9mm_16TPulley:3
- Mate:303: COTS_WCP-0783_1.125ODHexBearing:17 ↔ COTS_HTD5MM_9mm_16TPulley:4
- Flush:17: COTS_HTD5MM_9mm_16TPulley:3 ↔ COTS_HTD5MM_9mm_16TPulley:4
- Mate:304: COTS_WCP-0783_1.125ODHexBearing:17 ↔ COTS_HTD5MM_9mm_16TPulley:5
- Flush:18: COTS_HTD5MM_9mm_16TPulley:5 ↔ COTS_HTD5MM_9mm_16TPulley:6
- Mate:305: COTS_WCP-0783_1.125ODHexBearing:16 ↔ COTS_HTD5MM_9mm_16TPulley:6
- Mate:306: COTS_WCP-0783_1.125ODHexBearing:6 ↔ COTS_HTD5MM_9mm_16TPulley:7
- Mate:307: COTS_WCP-0783_1.125ODHexBearing:5 ↔ COTS_HTD5MM_9mm_16TPulley:8
- Flush:19: COTS_HTD5MM_9mm_16TPulley:7 ↔ COTS_HTD5MM_9mm_16TPulley:8
- Mate:308: COTS_WCP-0783_1.125ODHexBearing:11 ↔ COTS_HTD5MM_9mm_16TPulley:9
- Mate:309: COTS_WCP-0783_1.125ODHexBearing:19 ↔ COTS_HTD5MM_9mm_16TPulley:10
- Flush:20: COTS_HTD5MM_9mm_16TPulley:9 ↔ COTS_HTD5MM_9mm_16TPulley:10
- Mate:310: COTS_WCP-0783_1.125ODHexBearing:2 ↔ COTS_HTD5MM_9mm_16TPulley:12
- Mate:311: COTS_WCP-0783_1.125ODHexBearing:1 ↔ COTS_HTD5MM_9mm_16TPulley:11
- Flush:21: COTS_HTD5MM_9mm_16TPulley:11 ↔ COTS_HTD5MM_9mm_16TPulley:12
- Mate:312: COTS_WCP-0783_1.125ODHexBearing:26 ↔ COTS_HTD5MM_9mm_16TPulley:14
- Mate:313: COTS_WCP-0783_1.125ODHexBearing:12 ↔ COTS_HTD5MM_9mm_16TPulley:13
- Mate:314: COTS_WCP-0783_1.125ODHexBearing:15 ↔ COTS_HTD5MM_9mm_16TPulley:15
- Mate:315: COTS_WCP-0783_1.125ODHexBearing:15 ↔ COTS_HTD5MM_9mm_16TPulley:16
- Flush:22: COTS_HTD5MM_9mm_16TPulley:14 ↔ COTS_HTD5MM_9mm_16TPulley:16
- Flush:23: COTS_HTD5MM_9mm_16TPulley:13 ↔ COTS_HTD5MM_9mm_16TPulley:15
- Mate:316: COTS_WCP-0783_1.125ODHexBearing:12 ↔ COTS_HTD5MM_9mm_16TPulley:19
- Mate:317: COTS_WCP-0783_1.125ODHexBearing:13 ↔ COTS_HTD5MM_9mm_16TPulley:20
- Flush:24: COTS_HTD5MM_9mm_16TPulley:19 ↔ COTS_HTD5MM_9mm_16TPulley:20
- Mate:318: COTS_WCP-0783_1.125ODHexBearing:3 ↔ COTS_HTD5MM_9mm_16TPulley:17
- Mate:319: COTS_WCP-0783_1.125ODHexBearing:4 ↔ COTS_HTD5MM_9mm_16TPulley:18
- Flush:25: COTS_HTD5MM_9mm_16TPulley:17 ↔ COTS_HTD5MM_9mm_16TPulley:18
- Mate:320: COTS_WCP-0783_1.125ODHexBearing:27 ↔ COTS_90107A029_316 Stainless Steel Washer:17
- Mate:321: INDX_015_OuterHex:1 ↔ COTS_90107A029_316 Stainless Steel Washer:17
- Mate:322: INDX_015_OuterHex:1 ↔ COTS_0.25-20_ButtonHead_0.5inlong_StainlessSteel_92949A537:19
- Mate:323: COTS_90107A029_316 Stainless Steel Washer:17 ↔ COTS_0.25-20_ButtonHead_0.5inlong_StainlessSteel_92949A537:19
